# Autodesk Inventor assembly: Segment_Staender_v1
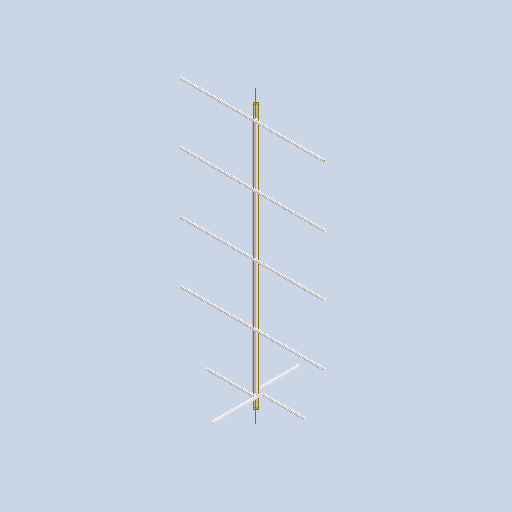
[picture p0: Inventor's stored thumbnail of the model, 512x512]
Saved by Autodesk Inventor 2025 (Build 290162000, 162)
## iProperties
Created: 2024-10-13
Part Number: Segment_Staender_v1
Document SubType Name: Assembly
Designer: Kai Altwicker
Author: Kai Altwicker
## iProperties of the stored document Klemmwinkelsatz_5.iam
Company: CADClick - www.CADClick.com
Created: 2024-10-10
Part Number: Klemmwinkelsatz_5
Description: STEP AP214
Document SubType Name: Assembly
Designer: Kai Altwicker
Authority: unknown authorization
Preprocessor: Spatial InterOp 3D
Title: cctmp_0BE804C5-1277-4A11-8FBA-5B98BBEA6A25_2024_10_10_16_06_07_0400_66932..stp
Author: KiM GmbH
Revision Number: NONE
## iProperties of the stored document item_0043784_Klemmwinkel 5_1.ipt
Created: 2024-10-17
Part Number: item_0043784_Klemmwinkel 5_1
Material: Generisch
Description: PART-item_0043784_Klemmwinkel 5_1-DESC
Document SubType Name: Modeling
Designer: Kai Altwicker
Density: 1 g/cm^3
Appearance: Vorgabe
Author: Kai Altwicker
Revision Number: NONE
## Documents named in this file (11)
- **C:\Users\Aldi\Repos\VolumanXR\hardware-capture\cad\rig_v1\Segment_Staender_v1.iam*LocalDocs*xAaaaacdaAaaaaaaaAaaaqbjxNf*Klemmwinkelsatz_5.iam
- **C:\Users\Aldi\Repos\VolumanXR\hardware-capture\cad\rig_v1\Segment_Staender_v1.iam*LocalDocs*xAaaaaqbaAaaaaaaaAaaaqrltHe*item_0043784_Klemmwinkel 5_1.ipt
- **C:\Users\tallA\Repos\VolumanXR\hardware-capture\cad\rig_v1\Segment_Staender_v1.iam*LocalDocs*xAaaaaqbaAaaaaaaaAaaaqrltHe*item_0043784_Klemmwinkel 5_1.ipt
- C:\Users\Aldi\Repos\VolumanXR\hardware-capture\cad\rig_v1\Segment_Staender_v1.iam
- C:\Users\Aldi\Repos\VolumanXR\hardware-capture\cad\Library\Profil_5_40x40_2500\Profil_5_40x40_2500\Profil_5_40x40_2500.ipt
- C:\Users\Aldi\Repos\VolumanXR\hardware-capture\cad\rig_v1\Profil_5_20x20_1500.ipt
- C:\Users\Aldi\Repos\VolumanXR\hardware-capture\cad\Library\Winkelsatz_20x20_einfach\Winkelsatz_20x20_einfach\Winkelsatz_20x20_einfach.ipt
- C:\Users\Aldi\Repos\VolumanXR\hardware-capture\cad\rig_v1\Profil_5_20x20_500.ipt
- C:\Users\Aldi\Repos\VolumanXR\hardware-capture\cad\dimensions.xlsx
- C:\Users\tallA\Repos\VolumanXR\hardware-capture\cad\dimensions.xlsx
- C:\Users\Aldi\Repos\VolumanXR\hardware-capture\cad\Library\Klemmwinkelsatz_5.step
## Components (25 placed, 5 different names)
1. Profil_5_40x40_2500:1 — Passend:4, Fluchtend:7, Passend:5, Fluchtend:11, Passend:7, Fluchtend:13, Passend:11, Fluchtend:14, Passend:14, Passend:15, Fluchtend:15, Fluchtend:16
2. Winkelsatz_20x20_einfach:1 — Passend:5, Passend:6, Fluchtend:10, Fluchtend:12
3. Profil_5_20x20_1500:1 — Passend:4, Fluchtend:7, Passend:6, Fluchtend:10, Fluchtend:11, Passend:8, Passend:9, Passend:10
4. Winkelsatz_20x20_einfach:2 — Passend:7, Passend:8, Fluchtend:12
5. Winkelsatz_20x20_einfach:3
6. Profil_5_20x20_1500:2
7. Winkelsatz_20x20_einfach:4
8. Winkelsatz_20x20_einfach:5
9. Profil_5_20x20_1500:3
10. Winkelsatz_20x20_einfach:6
11. Winkelsatz_20x20_einfach:7
12. Profil_5_20x20_1500:4
13. Winkelsatz_20x20_einfach:8
14. Profil_5_20x20_500:1 — Fluchtend:13, Passend:11, Fluchtend:14, Passend:12, Passend:13
15. Klemmwinkelsatz_5:2 [sub-assembly] — Passend:13, Passend:14, Fluchtend:16
16. Klemmwinkelsatz_5:1 [sub-assembly] — Passend:12, Passend:15, Fluchtend:15
17. Profil_5_20x20_500:2
18. Klemmwinkelsatz_5:3 [sub-assembly]
19. Klemmwinkelsatz_5:4 [sub-assembly]
20. Profil_5_20x20_500:3
21. Klemmwinkelsatz_5:5 [sub-assembly]
22. Klemmwinkelsatz_5:6 [sub-assembly]
23. Profil_5_20x20_500:4
24. Klemmwinkelsatz_5:7 [sub-assembly]
25. Klemmwinkelsatz_5:8 [sub-assembly]
## Component patterns: (4 elements, first: Winkelsatz_20x20_einfach:1 + Profil_5_20x20_1500:1 + Winkelsatz_20x20_einfach:2), (4 elements, first: Profil_5_20x20_500:1 + Klemmwinkelsatz_5:2 + Klemmwinkelsatz_5:1)
## Relationships (20: Mate 12, Flush 8)
- Passend:4 [Mate]: Profil_5_40x40_2500:1 ↔ Profil_5_20x20_1500:1
- Fluchtend:7 [Flush]: Profil_5_40x40_2500:1 ↔ Profil_5_20x20_1500:1
- Passend:5 [Mate]: Profil_5_40x40_2500:1 ↔ Winkelsatz_20x20_einfach:1
- Passend:6 [Mate]: Winkelsatz_20x20_einfach:1 ↔ Profil_5_20x20_1500:1
- Fluchtend:10 [Flush]: Winkelsatz_20x20_einfach:1 ↔ Profil_5_20x20_1500:1
- Fluchtend:11 [Flush] (-750 mm): Profil_5_40x40_2500:1 ↔ Profil_5_20x20_1500:1
- Passend:7 [Mate]: Profil_5_40x40_2500:1 ↔ Winkelsatz_20x20_einfach:2
- Passend:8 [Mate]: Profil_5_20x20_1500:1 ↔ Winkelsatz_20x20_einfach:2
- Fluchtend:12 [Flush]: Winkelsatz_20x20_einfach:1 ↔ Winkelsatz_20x20_einfach:2
- Passend:9 [Mate]: Profil_5_20x20_1500:1
- Passend:10 [Mate]: Profil_5_20x20_1500:1
- Fluchtend:13 [Flush]: Profil_5_40x40_2500:1 ↔ Profil_5_20x20_500:1
- Passend:11 [Mate]: Profil_5_40x40_2500:1 ↔ Profil_5_20x20_500:1
- Fluchtend:14 [Flush]: Profil_5_40x40_2500:1 ↔ Profil_5_20x20_500:1
- Passend:12 [Mate]: Profil_5_20x20_500:1 ↔ Klemmwinkelsatz_5:1
- Passend:13 [Mate]: Profil_5_20x20_500:1 ↔ Klemmwinkelsatz_5:2
- Passend:14 [Mate]: Profil_5_40x40_2500:1 ↔ Klemmwinkelsatz_5:2
- Passend:15 [Mate]: Profil_5_40x40_2500:1 ↔ Klemmwinkelsatz_5:1
- Fluchtend:15 [Flush] (2 mm): Profil_5_40x40_2500:1 ↔ Klemmwinkelsatz_5:1
- Fluchtend:16 [Flush] (2 mm): Profil_5_40x40_2500:1 ↔ Klemmwinkelsatz_5:2
## Named parameters: d_tol = 0.3 mm, d_wand = 1.5 mm, d_traeger = 625 mm, h_profil_20x20 = 20 mm, b_profil_40x40 = 40 mm, b_profil_20x20 = 20 mm, l_profil_20x20 = 1500 mm, l_profil_40x40 = 2500 mm, h_profil_40x40 = 40 mm, D_oct = 3621.32034 mm, D_dode = 8196.15242 mm, D_hexadeca = 7541.00924 mm, w_kamera_hori = 66 deg, w_kamera_vert = 41 deg, r_rasp_pi = 3 mm, b_rasp_pi = 56 mm, l_rasp_pi = 85 mm
